# Autodesk Inventor assembly: piston_sub_assembly
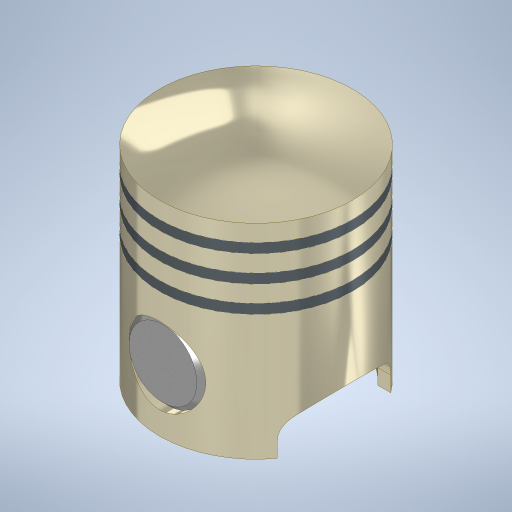
[picture p0: Inventor's stored thumbnail of the model, 512x512]
Saved by Autodesk Inventor 2023 (Build 270158000, 158)
## iProperties
Created: 2023-10-21
Part Number: piston_sub_assembly
Document SubType Name: Assembly
Designer: Beatrice
Author: Beatrice
## Documents named in this file (4)
- C:\Users\Beatrice\Documents\Inventor\4_Cylinder_Engine\4 cylinder engine assembly\piston_sub_assembly.iam
- C:\Users\Beatrice\Documents\Inventor\4_Cylinder_Engine\4 cylinder engine assembly\piston.ipt
- C:\Users\Beatrice\Documents\Inventor\4_Cylinder_Engine\4 cylinder engine assembly\piston_ring.ipt
- C:\Users\Beatrice\Documents\Inventor\4_Cylinder_Engine\4 cylinder engine assembly\piston_pin.ipt
## Components (5 placed, 3 different names)
1. piston:1 — Insert:1, Mate:1, Flush:1
2. piston_pin:1 — Mate:1, Flush:1
3. piston_ring:1 — Insert:1
4. piston_ring:2
5. piston_ring:3
## Component patterns: (3 elements, first: piston_ring:1)
## Relationships (3: Insert 1, Mate 1, Flush 1)
- Insert:1: piston:1 ↔ piston_ring:1
- Mate:1: piston:1 ↔ piston_pin:1
- Flush:1: piston:1 ↔ piston_pin:1
